# Autodesk Inventor assembly: 関節1_プーリ2個
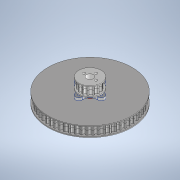
[picture p0: Inventor's stored thumbnail of the model, 180x180]
Saved by Autodesk Inventor 2021 (Build 250183000, 183)
## iProperties
Created: 2022-02-02
Part Number: 関節1_プーリ2個
Document SubType Name: Assembly
Designer: hirohumi
Author: hirohumi
## Documents named in this file (5)
- C:\Users\hirohumi\OneDrive\ドキュメント\ロボ研\2022NHKロボコン\R2_version1\3軸アーム\関節1_プーリ2個.iam
- C:\Users\hirohumi\OneDrive\ドキュメント\ロボ研\2022NHKロボコン\R2_version1\3軸アーム\プーリ_歯数60_関節1.ipt
- C:\Users\hirohumi\OneDrive\ドキュメント\ロボ研\2022NHKロボコン\R2_version1\3軸アーム\関節1_プーリ接続.ipt
- C:\Users\hirohumi\OneDrive\ドキュメント\ロボ研\2022NHKロボコン\R2_version1\3軸アーム\ベアリングフランジなし.ipt
- C:\Users\hirohumi\OneDrive\ドキュメント\ロボ研\2022NHKロボコン\R2_version1\3軸アーム\プーリ_歯数15.ipt
## Components (6 placed, 4 different names)
1. プーリ_歯数60_関節1:1 — 挿入:1, 挿入:2, 挿入:5
2. プーリ_歯数60_関節1:2 — 挿入:1, 挿入:2, 挿入:3, 挿入:4
3. 関節1_プーリ接続:1 — 挿入:3, 挿入:4, 挿入:8, 挿入:9
4. ベアリングフランジなし:1 — 挿入:5
5. プーリ_歯数15:1 — 挿入:6, 挿入:7, 挿入:8, 挿入:9
6. プーリ_歯数15:2 — 挿入:6, 挿入:7
## Relationships (9: Insert 9)
- 挿入:1 [Insert]: プーリ_歯数60_関節1:1 ↔ プーリ_歯数60_関節1:2
- 挿入:2 [Insert]: プーリ_歯数60_関節1:1 ↔ プーリ_歯数60_関節1:2
- 挿入:3 [Insert]: プーリ_歯数60_関節1:2 ↔ 関節1_プーリ接続:1
- 挿入:4 [Insert]: プーリ_歯数60_関節1:2 ↔ 関節1_プーリ接続:1
- 挿入:5 [Insert]: プーリ_歯数60_関節1:1 ↔ ベアリングフランジなし:1
- 挿入:6 [Insert]: プーリ_歯数15:1 ↔ プーリ_歯数15:2
- 挿入:7 [Insert]: プーリ_歯数15:1 ↔ プーリ_歯数15:2
- 挿入:8 [Insert]: 関節1_プーリ接続:1 ↔ プーリ_歯数15:1
- 挿入:9 [Insert]: 関節1_プーリ接続:1 ↔ プーリ_歯数15:1
